# Autodesk Inventor assembly: WATCHY_CUT
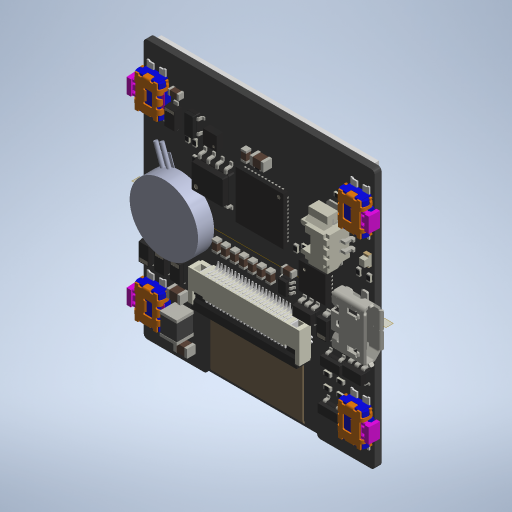
[picture p0: Inventor's stored thumbnail of the model, 512x512]
Saved by Autodesk Inventor 2023 (Build 270158000, 158)
## iProperties
Company: SQFMI
Created: 2020-12-31
Part Number: WATCHY_CUT
Description: KiCad electronic assembly
Document SubType Name: Assembly
Designer: nigel
Authority: Unknown
Sending System: KiCad to STEP converter
Preprocessor: Open CASCADE STEP processor 6.9
Title: Watchy.step
Author: SQFMI
## Documents named in this file (22)
- D:\NIGEL\Documents\GitHub\Watchy-CAD\CAD\Base Model\WATCHY_CUT_TC.iam
- D:\NIGEL\Documents\GitHub\Watchy-CAD\CAD\Base Model\USB_Micro-B_Molex_47346-0001.iam
- D:\NIGEL\Documents\GitHub\Watchy-CAD\CAD\Base Model\C_0603_1608Metric.iam
- D:\NIGEL\Documents\GitHub\Watchy-CAD\CAD\Base Model\Button.iam
- D:\NIGEL\Documents\GitHub\Watchy-CAD\CAD\Base Model\LGA-12_2x2mm_P0.5mm.iam
- D:\NIGEL\Documents\GitHub\Watchy-CAD\CAD\Base Model\FPC-24.iam
- D:\NIGEL\Documents\GitHub\Watchy-CAD\CAD\Base Model\Molex_PicoBlade_53261-0271_1x02-1MP_P1.25mm_Horizontal.iam
- D:\NIGEL\Documents\GitHub\Watchy-CAD\CAD\Base Model\R_0402_1005Metric.iam
- D:\NIGEL\Documents\GitHub\Watchy-CAD\CAD\Base Model\QFN-24-1EP_4x4mm_P0.5mm_EP2.7x2.7mm.iam
- D:\NIGEL\Documents\GitHub\Watchy-CAD\CAD\Base Model\C_0805_2012Metric.iam
- D:\NIGEL\Documents\GitHub\Watchy-CAD\CAD\Base Model\D_SOD-123.iam
- D:\NIGEL\Documents\GitHub\Watchy-CAD\CAD\Base Model\LED_0603_1608Metric.iam
- D:\NIGEL\Documents\GitHub\Watchy-CAD\CAD\Base Model\D_SOD-123F.iam
- D:\NIGEL\Documents\GitHub\Watchy-CAD\CAD\Base Model\L_1210_3225Metric.iam
- D:\NIGEL\Documents\GitHub\Watchy-CAD\CAD\Base Model\SOT-23.iam
- D:\NIGEL\Documents\GitHub\Watchy-CAD\CAD\Base Model\QFN-48-1EP_7x7mm_P0.5mm_EP5.15x5.15mm.iam
- D:\NIGEL\Documents\GitHub\Watchy-CAD\CAD\Base Model\SOT-23-5.iam
- D:\NIGEL\Documents\GitHub\Watchy-CAD\CAD\Base Model\SOT-363_SC-70-6.iam
- D:\NIGEL\Documents\GitHub\Watchy-CAD\CAD\Base Model\SOIC-8_3.9x4.9mm_P1.27mm.iam
- D:\NIGEL\Documents\GitHub\Watchy-CAD\CAD\Base Model\PagerMotor.iam
- D:\NIGEL\Documents\GitHub\Watchy-CAD\CAD\Base Model\COMPOUND_SMALL.ipt
- D:\NIGEL\Documents\GitHub\Watchy-CAD\CAD\Base Model\Display_Touchscreen.iam
## Components (55 placed, 21 different names)
1. USB_Micro-B_Molex_47346-0001:1 [sub-assembly]
2. C_0603_1608Metric:1 [sub-assembly]
3. Button:1 [sub-assembly]
4. Button:2 [sub-assembly]
5. Button:3 [sub-assembly]
6. Button:4 [sub-assembly]
7. LGA-12_2x2mm_P0.5mm:1 [sub-assembly]
8. FPC-24:1 [sub-assembly]
9. Molex_PicoBlade_53261-0271_1x02-1MP_P1.25mm_Horizontal:1 [sub-assembly]
10. R_0402_1005Metric:1 [sub-assembly]
11. QFN-24-1EP_4x4mm_P0.5mm_EP2.7x2.7mm:1 [sub-assembly]
12. R_0402_1005Metric:2 [sub-assembly]
13. C_0603_1608Metric:2 [sub-assembly]
14. Display_Touchscreen:1 [sub-assembly] — Mate:1, Flush:1, Flush:2
15. C_0603_1608Metric:3 [sub-assembly]
16. C_0603_1608Metric:4 [sub-assembly]
17. C_0805_2012Metric:1 [sub-assembly]
18. C_0805_2012Metric:2 [sub-assembly]
19. C_0603_1608Metric:5 [sub-assembly]
20. C_0603_1608Metric:6 [sub-assembly]
21. C_0603_1608Metric:7 [sub-assembly]
22. C_0603_1608Metric:8 [sub-assembly]
23. C_0603_1608Metric:9 [sub-assembly]
24. C_0603_1608Metric:10 [sub-assembly]
25. C_0805_2012Metric:3 [sub-assembly]
26. D_SOD-123:1 [sub-assembly]
27. D_SOD-123:2 [sub-assembly]
28. D_SOD-123:3 [sub-assembly]
29. D_SOD-123:4 [sub-assembly]
30. LED_0603_1608Metric:1 [sub-assembly]
31. D_SOD-123F:1 [sub-assembly]
32. L_1210_3225Metric:1 [sub-assembly]
33. SOT-23:1 [sub-assembly]
34. SOT-23:2 [sub-assembly]
35. SOT-23:3 [sub-assembly]
36. R_0402_1005Metric:3 [sub-assembly]
37. R_0402_1005Metric:4 [sub-assembly]
38. R_0402_1005Metric:5 [sub-assembly]
39. R_0402_1005Metric:6 [sub-assembly]
40. R_0402_1005Metric:7 [sub-assembly]
41. R_0402_1005Metric:8 [sub-assembly]
42. R_0402_1005Metric:9 [sub-assembly]
43. R_0402_1005Metric:10 [sub-assembly]
44. R_0402_1005Metric:11 [sub-assembly]
45. R_0402_1005Metric:13 [sub-assembly]
46. R_0402_1005Metric:14 [sub-assembly]
47. R_0402_1005Metric:15 [sub-assembly]
48. QFN-48-1EP_7x7mm_P0.5mm_EP5.15x5.15mm:1 [sub-assembly]
49. SOT-23-5:1 [sub-assembly]
50. SOT-23-5:2 [sub-assembly]
51. SOT-363_SC-70-6:1 [sub-assembly]
52. SOIC-8_3.9x4.9mm_P1.27mm:1 [sub-assembly]
53. R_0402_1005Metric:16 [sub-assembly]
54. PagerMotor:1 [sub-assembly]
55. COMPOUND (2):1 — Mate:1, Flush:1, Flush:2
## Relationships (3: Flush 2, Mate 1)
- Mate:1: Display_Touchscreen:1 ↔ COMPOUND (2):1
- Flush:1 (1.4 mm): Display_Touchscreen:1 ↔ COMPOUND (2):1
- Flush:2 (0.4 mm): Display_Touchscreen:1 ↔ COMPOUND (2):1
